# Autodesk Inventor assembly: Assembly1
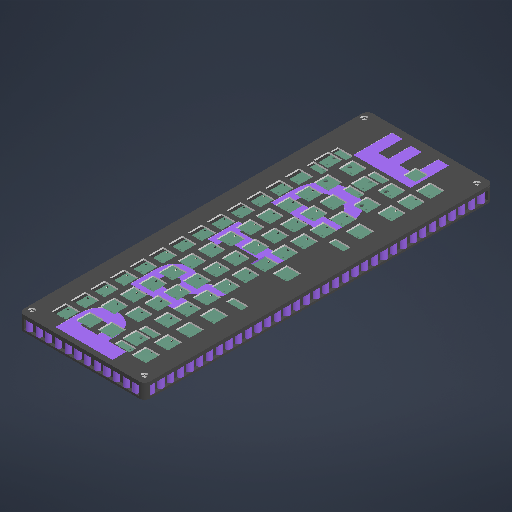
[picture p0: Inventor's stored thumbnail of the model, 512x512]
Saved by Autodesk Inventor 2026 (Build 300175050, 175E)
## iProperties
Created: 2025-07-05
Part Number: Assembly1
Document SubType Name: Assembly
Designer: SaiAn
Author: SaiAn
## Documents named in this file (4)
- C:\Full-Split Keyboard\Assembly1.iam
- C:\Full-Split Keyboard\Top_Plate_Mkey.ipt
- C:\Full-Split Keyboard\Bottom_Plate_MKey.ipt
- C:\Full-Split Keyboard\FullSplit_Keyboard_PCB\FullSplit_Keyboard_PCB\FullSplit_Keyboard_PCB\FullSplit_Keyboard_PCB.iam
## Components (3 placed, 3 different names)
1. Top_Plate_Mkey:1 — Mate:4, Flush:1, Flush:2
2. Bottom_Plate_MKey:1 — Mate:1, Mate:2, Mate:3, Mate:4, Flush:1, Flush:2
3. FullSplit_Keyboard_PCB:1 [sub-assembly] — Mate:1, Mate:2, Mate:3
## Relationships (6: Mate 4, Flush 2)
- Mate:1: Bottom_Plate_MKey:1 ↔ FullSplit_Keyboard_PCB:1
- Mate:2: Bottom_Plate_MKey:1 ↔ FullSplit_Keyboard_PCB:1
- Mate:3: Bottom_Plate_MKey:1 ↔ FullSplit_Keyboard_PCB:1
- Mate:4: Top_Plate_Mkey:1 ↔ Bottom_Plate_MKey:1
- Flush:1: Top_Plate_Mkey:1 ↔ Bottom_Plate_MKey:1
- Flush:2: Top_Plate_Mkey:1 ↔ Bottom_Plate_MKey:1
